# Autodesk Inventor assembly: 217-3269-3CIM-WCD_orient2
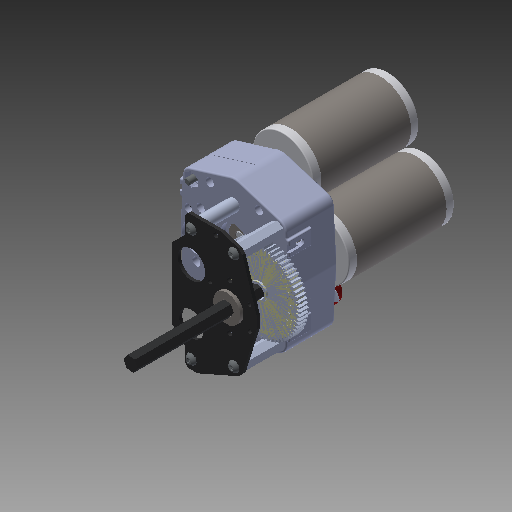
[picture p0: Inventor's stored thumbnail of the model, 512x512]
Saved by Autodesk Inventor 2017 (Build 210142000, 142)
## iProperties
Created: 2015-12-17
Part Number: 217-3269-3CIM-WCD_orient2
Description: STEP AP214
Document SubType Name: Assembly
Designer: rickab1
Sending System: SolidWorks 2015
Preprocessor: SwSTEP 2.0
Title: 217-3269-3CIM-WCD
Revision Number: ANY
## Documents named in this file (51)
- C:\Users\FIRSTUser\Documents\GrabCAD\2017 Robot\Imported Components\Gearboxes\3CIM Ball Shift WCD\217-3269-3CIM-WCD_orient2.iam
- 217-3269-3CIM-WCD_orient1.iam
- C:\Users\FIRSTUser\Documents\GrabCAD\2017 Robot\Imported Components\Gearboxes\3CIM Ball Shift WCD\217-2733-001 Rev2.ipt
- C:\Users\FIRSTUser\Documents\GrabCAD\2017 Robot\Imported Components\Gearboxes\3CIM Ball Shift WCD\217-2731-001 Rev2.ipt
- C:\Users\FIRSTUser\Documents\GrabCAD\2017 Robot\Imported Components\Gearboxes\3CIM Ball Shift WCD\217-2789-001 Rev2.ipt
- C:\Users\FIRSTUser\Documents\GrabCAD\2017 Robot\Imported Components\Gearboxes\3CIM Ball Shift WCD\217-2778-001 Rev2_NCQ8A075-050M.iam
- C:\Users\FIRSTUser\Documents\GrabCAD\2017 Robot\Imported Components\Gearboxes\3CIM Ball Shift WCD\217-2428-012 Rev2.ipt
- C:\Users\FIRSTUser\Documents\GrabCAD\2017 Robot\Imported Components\Gearboxes\3CIM Ball Shift WCD\217-2428-005 Rev1.ipt
- C:\Users\FIRSTUser\Documents\GrabCAD\2017 Robot\Imported Components\Gearboxes\3CIM Ball Shift WCD\SCREW-832-0375.ipt
- C:\Users\FIRSTUser\Documents\GrabCAD\2017 Robot\Imported Components\Gearboxes\3CIM Ball Shift WCD\SBS1_SBS-0632-0250.ipt
- C:\Users\FIRSTUser\Documents\GrabCAD\2017 Robot\Imported Components\Gearboxes\3CIM Ball Shift WCD\217-4098-100 Rev1.iam
- C:\Users\FIRSTUser\Documents\GrabCAD\2017 Robot\Imported Components\Gearboxes\3CIM Ball Shift WCD\217-2428-017 Rev2.ipt
- C:\Users\FIRSTUser\Documents\GrabCAD\2017 Robot\Imported Components\Gearboxes\3CIM Ball Shift WCD\217-2428-016 Rev3_Spur01.ipt
- C:\Users\FIRSTUser\Documents\GrabCAD\2017 Robot\Imported Components\Gearboxes\3CIM Ball Shift WCD\217-2428-019 Rev1.ipt
- C:\Users\FIRSTUser\Documents\GrabCAD\2017 Robot\Imported Components\Gearboxes\3CIM Ball Shift WCD\217-2428-006 Rev1.ipt
- C:\Users\FIRSTUser\Documents\GrabCAD\2017 Robot\Imported Components\Gearboxes\3CIM Ball Shift WCD\217-2614-001_12t.ipt
- C:\Users\FIRSTUser\Documents\GrabCAD\2017 Robot\Imported Components\Gearboxes\3CIM Ball Shift WCD\217-2761-001 rev1.ipt
- C:\Users\FIRSTUser\Documents\GrabCAD\2017 Robot\Imported Components\Gearboxes\3CIM Ball Shift WCD\217-3195-002 rev2.ipt
- C:\Users\FIRSTUser\Documents\GrabCAD\2017 Robot\Imported Components\Gearboxes\3CIM Ball Shift WCD\217-3195-001 Rev1.ipt
- C:\Users\FIRSTUser\Documents\GrabCAD\2017 Robot\Imported Components\Gearboxes\3CIM Ball Shift WCD\Nylock Nut_NNY2520-ZC.ipt
- C:\Users\FIRSTUser\Documents\GrabCAD\2017 Robot\Imported Components\Gearboxes\3CIM Ball Shift WCD\276-1027-001.ipt
- C:\Users\FIRSTUser\Documents\GrabCAD\2017 Robot\Imported Components\Gearboxes\3CIM Ball Shift WCD\SCREW-832-1750.ipt
- C:\Users\FIRSTUser\Documents\GrabCAD\2017 Robot\Imported Components\Gearboxes\3CIM Ball Shift WCD\217-2428-004 Rev3.ipt
- C:\Users\FIRSTUser\Documents\GrabCAD\2017 Robot\Imported Components\Gearboxes\3CIM Ball Shift WCD\SBS1_SBS-2520-1625SS.ipt
- C:\Users\FIRSTUser\Documents\GrabCAD\2017 Robot\Imported Components\Gearboxes\3CIM Ball Shift WCD\SBS1_SBS2520-1750.ipt
- C:\Users\FIRSTUser\Documents\GrabCAD\2017 Robot\Imported Components\Gearboxes\3CIM Ball Shift WCD\217-2428-021 Rev1.ipt
- C:\Users\FIRSTUser\Documents\GrabCAD\2017 Robot\Imported Components\Gearboxes\3CIM Ball Shift WCD\217-2428-029 Rev1.ipt
- C:\Users\FIRSTUser\Documents\GrabCAD\2017 Robot\Imported Components\Gearboxes\3CIM Ball Shift WCD\Grayhill Lock Washer.ipt
- C:\Users\FIRSTUser\Documents\GrabCAD\2017 Robot\Imported Components\Gearboxes\3CIM Ball Shift WCD\Grayhill Nut.ipt
- C:\Users\FIRSTUser\Documents\GrabCAD\2017 Robot\Imported Components\Gearboxes\3CIM Ball Shift WCD\217-2000.ipt
- C:\Users\FIRSTUser\Documents\GrabCAD\2017 Robot\Imported Components\Gearboxes\3CIM Ball Shift WCD\Grahill Encoder.ipt
- C:\Users\FIRSTUser\Documents\GrabCAD\2017 Robot\Imported Components\Gearboxes\3CIM Ball Shift WCD\217-3195-009 Rev1_wcd 2.ipt
- C:\Users\FIRSTUser\Documents\GrabCAD\2017 Robot\Imported Components\Gearboxes\3CIM Ball Shift WCD\217-3195-006 Rev1_WCD.ipt
- C:\Users\FIRSTUser\Documents\GrabCAD\2017 Robot\Imported Components\Gearboxes\3CIM Ball Shift WCD\SBS1_SBS-2520-2250.ipt
- C:\Users\FIRSTUser\Documents\GrabCAD\2017 Robot\Imported Components\Gearboxes\3CIM Ball Shift WCD\SBS1_SBS2520-0625ZC.ipt
- C:\Users\FIRSTUser\Documents\GrabCAD\2017 Robot\Imported Components\Gearboxes\3CIM Ball Shift WCD\217-3195-003 rev2.ipt
- C:\Users\FIRSTUser\Documents\GrabCAD\2017 Robot\Imported Components\Gearboxes\3CIM Ball Shift WCD\217-2617-003 Rev1.ipt
- C:\Users\FIRSTUser\Documents\GrabCAD\2017 Robot\Imported Components\Gearboxes\3CIM Ball Shift WCD\217-3109-001 Rev1.ipt
- C:\Users\FIRSTUser\Documents\GrabCAD\2017 Robot\Imported Components\Gearboxes\3CIM Ball Shift WCD\217-2734-001 Rev3.ipt
- C:\Users\FIRSTUser\Documents\GrabCAD\2017 Robot\Imported Components\Gearboxes\3CIM Ball Shift WCD\217-2617-004 Rev1_97431A340_grv.ipt
- C:\Users\FIRSTUser\Documents\GrabCAD\2017 Robot\Imported Components\Gearboxes\3CIM Ball Shift WCD\217-2702-001_20t.ipt
- C:\Users\FIRSTUser\Documents\GrabCAD\2017 Robot\Imported Components\Gearboxes\3CIM Ball Shift WCD\217-2715-002 Rev1_64t.ipt
- C:\Users\FIRSTUser\Documents\GrabCAD\2017 Robot\Imported Components\Gearboxes\3CIM Ball Shift WCD\217-2704-001_24.ipt
- C:\Users\FIRSTUser\Documents\GrabCAD\2017 Robot\Imported Components\Gearboxes\3CIM Ball Shift WCD\217-2714-002 Rev1_60t.ipt
- C:\Users\FIRSTUser\Documents\GrabCAD\2017 Robot\Imported Components\Gearboxes\3CIM Ball Shift WCD\217-3221-002 Rev1.ipt
- C:\Users\FIRSTUser\Documents\GrabCAD\2017 Robot\Imported Components\Gearboxes\3CIM Ball Shift WCD\217-2705-001_30t.ipt
- C:\Users\FIRSTUser\Documents\GrabCAD\2017 Robot\Imported Components\Gearboxes\3CIM Ball Shift WCD\217-2712-002 Rev1_50t.ipt
- C:\Users\FIRSTUser\Documents\GrabCAD\2017 Robot\Imported Components\Gearboxes\3CIM Ball Shift WCD\217-2706-001_34t.ipt
- C:\Users\FIRSTUser\Documents\GrabCAD\2017 Robot\Imported Components\Gearboxes\3CIM Ball Shift WCD\217-3288-001 Rev3.iam
- C:\Users\FIRSTUser\Documents\GrabCAD\2017 Robot\Imported Components\Gearboxes\3CIM Ball Shift WCD\217-3210-001 Rev1_30t.ipt
- C:\Users\FIRSTUser\Documents\GrabCAD\2017 Robot\Imported Components\Gearboxes\3CIM Ball Shift WCD\217-2711-002 Rev1_50t.ipt
## Components (80 placed, 80 different names)
1. 217-2733-001 Rev2_1
2. 217-2733-001 Rev2_2
3. 217-2731-001 Rev2_3
4. 217-2789-001 Rev2_4
5. 217-2778-001 Rev2_NCQ8A075-050M_5 [sub-assembly]
6. 217-2428-012 Rev2_6
7. 217-2428-005 Rev1_7
8. 217-2428-005 Rev1_8
9. SCREW-832-0375_9
10. SCREW-832-0375_10
11. SCREW-832-0375_11
12. SCREW-832-0375_12
13. SBS1_SBS-0632-0250_13
14. SBS1_SBS-0632-0250_14
15. 217-4098-100 Rev1_15 [sub-assembly]
16. 217-2428-017 Rev2_16
17. 217-2428-016 Rev3_Spur01_17
18. 217-2428-019 Rev1_18
19. 217-2428-006 Rev1_19
20. 217-2428-006 Rev1_20
21. SCREW-832-0375_21
22. SCREW-832-0375_22
23. SCREW-832-0375_23
24. SCREW-832-0375_24
25. 217-2614-001_12t_25
26. 217-2761-001 rev1_26
27. 217-2761-001 rev1_27
28. 217-2614-001_12t_28
29. 217-2614-001_12t_29
30. 217-2761-001 rev1_30
31. 217-3195-002 rev2_31 — Mate:6, Mate:8, Mate:10, Mate:11, Mate:24, Mate:25
32. 217-3195-001 Rev1_32
33. Nylock Nut_NNY2520-ZC_33
34. Nylock Nut_NNY2520-ZC_34
35. Nylock Nut_NNY2520-ZC_35
36. 276-1027-001_36
37. 276-1027-001_37
38. SCREW-832-1750_38
39. SCREW-832-1750_39
40. Nylock Nut_NNY2520-ZC_40
41. 217-2428-004 Rev3_41
42. SBS1_SBS-2520-1625SS_42
43. SBS1_SBS-2520-1625SS_43
44. SBS1_SBS2520-1750_44
45. SBS1_SBS2520-1750_45
46. 217-2428-021 Rev1_46
47. 217-2428-029 Rev1_47
48. Grayhill Lock Washer_48
49. Grayhill Nut_49
50. 217-2000_50
51. 217-2000_51
52. 217-2000_52
53. Grahill Encoder_53
54. 217-3195-009 Rev1_wcd 2_54 — Mate:5
55. 217-3195-006 Rev1_WCD_55 — Mate:6, Mate:7, Mate:8, Mate:13
56. 217-3195-009 Rev1_wcd 2_56 — Mate:4
57. 217-3195-006 Rev1_WCD_57 — Mate:9, Mate:10, Mate:11, Mate:12
58. Nylock Nut_NNY2520-ZC_58
59. Nylock Nut_NNY2520-ZC_59
60. SBS1_SBS-2520-2250_60
61. SBS1_SBS2520-0625ZC_61 — Mate:13, Mate:14
62. SBS1_SBS2520-0625ZC_62 — Mate:12, Mate:15
63. SBS1_SBS-2520-2250_63 — Mate:3
64. 217-3195-003 rev2_64 — Mate:1, Mate:2, Mate:3, Mate:4, Mate:5, Mate:7, Mate:9, Mate:14, Mate:15
65. 217-2617-003 Rev1_65 — Mate:20, Mate:21, Mate:22, Mate:23
66. 217-3109-001 Rev1_66 — Mate:22, Mate:23, Mate:24, Mate:25
67. 217-2734-001 Rev3_67 — Mate:1, Mate:2
68. 217-2617-004 Rev1_97431A340_grv_68 — Mate:20, Mate:21, Mate:26
69. 217-2617-004 Rev1_97431A340_grv_69
70. 217-2702-001_20t_70
71. 217-2715-002 Rev1_64t_71 — Mate:16, Flush:2
72. 217-2704-001_24_72
73. 217-2714-002 Rev1_60t_73 — Mate:16, Mate:18, Mate:19, Flush:1, Flush:2, Flush:3, Mate:26
74. 217-3221-002 Rev1_74 — Mate:18, Flush:3
75. 217-2705-001_30t_75
76. 217-2712-002 Rev1_50t_76 — Mate:19, Flush:1
77. 217-2706-001_34t_77
78. 217-3288-001 Rev3_78 [sub-assembly]
79. 217-3210-001 Rev1_30t_79
80. 217-2711-002 Rev1_50t_80
## Relationships (28: Mate 25, Flush 3)
- Mate:1: 217-3195-003 rev2_64 ↔ 217-2734-001 Rev3_67
- Mate:2: 217-3195-003 rev2_64 ↔ 217-2734-001 Rev3_67
- Mate:3: SBS1_SBS-2520-2250_63 ↔ 217-3195-003 rev2_64
- Mate:4: 217-3195-009 Rev1_wcd 2_56 ↔ 217-3195-003 rev2_64
- Mate:5: 217-3195-009 Rev1_wcd 2_54 ↔ 217-3195-003 rev2_64
- Mate:6: 217-3195-002 rev2_31 ↔ 217-3195-006 Rev1_WCD_55
- Mate:7: 217-3195-006 Rev1_WCD_55 ↔ 217-3195-003 rev2_64
- Mate:8: 217-3195-002 rev2_31 ↔ 217-3195-006 Rev1_WCD_55
- Mate:9: 217-3195-006 Rev1_WCD_57 ↔ 217-3195-003 rev2_64
- Mate:10: 217-3195-002 rev2_31 ↔ 217-3195-006 Rev1_WCD_57
- Mate:11: 217-3195-002 rev2_31 ↔ 217-3195-006 Rev1_WCD_57
- Mate:12: 217-3195-006 Rev1_WCD_57 ↔ SBS1_SBS2520-0625ZC_62
- Mate:13: 217-3195-006 Rev1_WCD_55 ↔ SBS1_SBS2520-0625ZC_61
- Mate:14: SBS1_SBS2520-0625ZC_61 ↔ 217-3195-003 rev2_64
- Mate:15: SBS1_SBS2520-0625ZC_62 ↔ 217-3195-003 rev2_64
- Mate:16: 217-2715-002 Rev1_64t_71 ↔ 217-2714-002 Rev1_60t_73
- Mate:18: 217-2714-002 Rev1_60t_73 ↔ 217-3221-002 Rev1_74
- Mate:19: 217-2714-002 Rev1_60t_73 ↔ 217-2712-002 Rev1_50t_76
- Flush:1: 217-2714-002 Rev1_60t_73 ↔ 217-2712-002 Rev1_50t_76
- Flush:2: 217-2715-002 Rev1_64t_71 ↔ 217-2714-002 Rev1_60t_73
- Flush:3: 217-2714-002 Rev1_60t_73 ↔ 217-3221-002 Rev1_74
- Mate:20: 217-2617-003 Rev1_65 ↔ 217-2617-004 Rev1_97431A340_grv_68
- Mate:21: 217-2617-003 Rev1_65 ↔ 217-2617-004 Rev1_97431A340_grv_68
- Mate:22: 217-2617-003 Rev1_65 ↔ 217-3109-001 Rev1_66
- Mate:23: 217-2617-003 Rev1_65 ↔ 217-3109-001 Rev1_66
- Mate:24: 217-3195-002 rev2_31 ↔ 217-3109-001 Rev1_66
- Mate:25: 217-3195-002 rev2_31 ↔ 217-3109-001 Rev1_66
- Mate:26: 217-2617-004 Rev1_97431A340_grv_68 ↔ 217-2714-002 Rev1_60t_73
